# Autodesk Inventor assembly: CentralBeam1of2
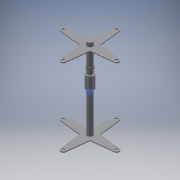
[picture p0: Inventor's stored thumbnail of the model, 180x180]
Saved by Autodesk Inventor 2016 SP1 (Build 200210100, 210)
## iProperties
Created: 2016-07-04
Part Number: CentralBeam1of2
Document SubType Name: Assembly
Designer: Tore Den Store
Author: Tore Den Store
## Documents named in this file (3)
- C:\Users\Jonatan\Documents\Inventor\Vertical axis wind turbine\WindPartCentral\CentralBeam1of2.iam
- C:\Users\Jonatan\Documents\Inventor\Vertical axis wind turbine\WindPartCentral\WindCentralbeam.ipt
- C:\Users\Jonatan\Documents\Inventor\Vertical axis wind turbine\WindPartCentral\1-of-4-part holder.ipt
## Components (3 placed, 2 different names)
1. WindCentralbeam:1 — Mate:1, Mate:2, Mate:3, Mate:4
2. 1-of-4-part holder:1 — Mate:1, Mate:2
3. 1-of-4-part holder:2 — Mate:3, Mate:4
## Relationships (4: Mate 4)
- Mate:1: WindCentralbeam:1 ↔ 1-of-4-part holder:1
- Mate:2: WindCentralbeam:1 ↔ 1-of-4-part holder:1
- Mate:3: WindCentralbeam:1 ↔ 1-of-4-part holder:2
- Mate:4: WindCentralbeam:1 ↔ 1-of-4-part holder:2
